# Autodesk Inventor assembly: capacitor_MIR
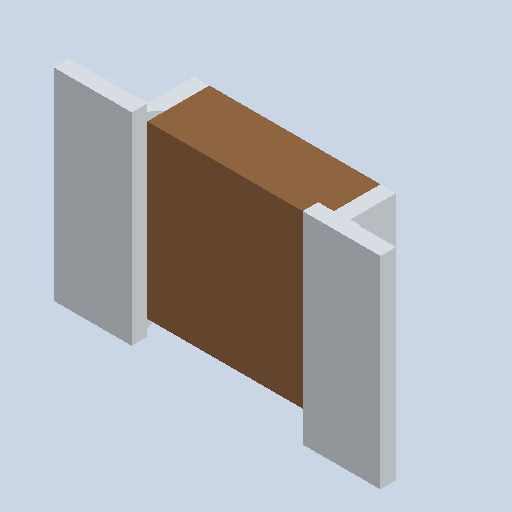
[picture p0: Inventor's stored thumbnail of the model, 512x512]
Saved by Autodesk Inventor 2025 (Build 290162000, 162)
## iProperties
Created: 2025-09-09
Part Number: capacitor_MIR
Document SubType Name: Assembly
Designer: jirne
Author: jirne
## Documents named in this file (3)
- C:\Users\jirne\JVR11\hardware\library\3D\DCJ11\capacitor\capacitor_MIR.iam
- C:\Users\jirne\JVR11\hardware\library\3D\DCJ11\capacitor\body_MIR.ipt
- C:\Users\jirne\JVR11\hardware\library\3D\DCJ11\capacitor\connection_MIR.ipt
## Components (3 placed, 2 different names)
1. body_MIR:1 — Mate:2, Mate:1, Mate:4, Mate:3
2. connection_MIR:1 — Mate:2, Mate:1
3. connection_MIR:2 — Mate:4, Mate:3
## Relationships (4: Mate 4)
- Mate:2: body_MIR:1 ↔ connection_MIR:1
- Mate:1: body_MIR:1 ↔ connection_MIR:1
- Mate:4: body_MIR:1 ↔ connection_MIR:2
- Mate:3: body_MIR:1 ↔ connection_MIR:2
